# Autodesk Inventor assembly: Handle_Assembly
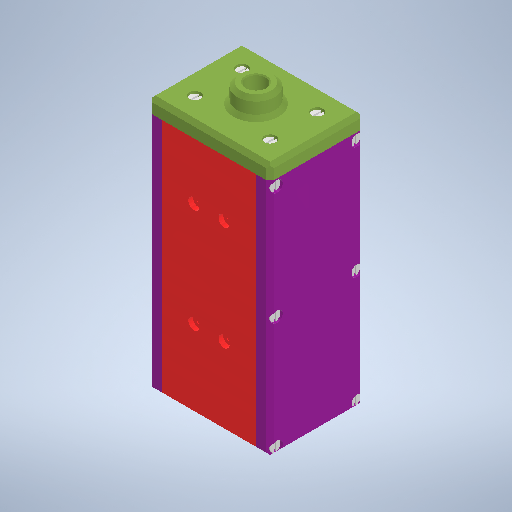
[picture p0: Inventor's stored thumbnail of the model, 512x512]
Saved by Autodesk Inventor 2026.2 (Build 302298010, 298A)
## iProperties
Created: 2026-05-07
Part Number: Handle_Assembly
Document SubType Name: Assembly
Designer: piete
Author: piete
## Documents named in this file (9)
- C:\Users\piete\Desktop\Skripsie\Documents\Detail Design\Handle Design\Handle_Assembly.iam
- C:\Users\piete\Desktop\Skripsie\Documents\Detail Design\Handle Design\Main_Cover.ipt
- C:\Users\piete\Desktop\Skripsie\Documents\Detail Design\Handle Design\Front_Cover.ipt
- C:\Users\piete\Desktop\Skripsie\Documents\Detail Design\Handle Design\Top_Covers.ipt
- C:\Users\piete\Desktop\Skripsie\Documents\Detail Design\Handle Design\Heat_Inserts.ipt
- C:\Users\piete\OneDrive\Documents\Inventor\Content Center Files\R2026\en-US\ISO 2009(2)\ISO 2009 - M3 x 20 - 17,35 - ISO.ipt
- C:\Users\piete\OneDrive\Documents\Inventor\Content Center Files\R2026\en-US\ISO 4036(2)\ISO 4036 - M3(2).ipt
- C:\Users\piete\OneDrive\Documents\Inventor\Content Center Files\R2026\en-US\ISO 2009(2)\ISO 2009 - M3 x 10 - 7,35 - ISO.ipt
- C:\Users\piete\Desktop\Skripsie\Documents\Detail Design\RS Components\186106 QS-G1_8-4-I.ipt
## Components (38 placed, 8 different names)
1. Main_Cover:1 — Mate:4, Mate:5, Mate:6, Flush:1, Mate:8, Flush:2, Mate:9, Flush:8, Mate:11, Mate:12, Mate:13, Mate:14, Mate:15, Mate:16, Flush:14, Mate:17, Mate:18, Mate:19, Mate:20, Mate:21, Mate:22, Mate:28, Mate:30, Mate:32, Mate:34, Mate:47, Mate:48, Mate:49, Mate:50
2. Front_Cover:1 — Mate:4, Mate:5, Mate:6, Mate:7, Mate:10, Mate:23, Mate:24, Mate:25, Mate:26, Flush:15, Flush:16, Flush:17, Flush:18, Angle:1, Angle:2
3. Top_Covers:1 — Flush:2, Mate:9, Mate:10, Mate:35, Mate:36, Mate:37, Mate:38, Mate:39, Mate:40, Flush:26
4. Top_Covers:2 — Flush:1, Mate:7, Mate:8, Flush:32, Mate:41, Mate:42, Mate:43, Mate:44, Mate:45, Mate:46
5. Heat_Inserts:1 — Flush:7, Flush:8, Mate:14
6. Heat_Inserts:2 — Flush:6, Flush:7, Mate:16
7. Heat_Inserts:3 — Flush:5, Flush:6, Mate:15
8. Heat_Inserts:4 — Flush:4, Flush:5, Mate:12
9. Heat_Inserts:5 — Flush:3, Mate:11
10. Heat_Inserts:6 — Flush:3, Flush:4, Mate:13
11. Heat_Inserts:7 — Flush:10, Mate:17
12. Heat_Inserts:8 — Flush:11, Mate:18
13. Heat_Inserts:9 — Flush:12, Flush:13, Mate:22
14. Heat_Inserts:10 — Flush:9, Flush:11, Flush:14, Mate:20
15. Heat_Inserts:11 — Flush:9, Flush:10, Flush:12, Mate:19
16. Heat_Inserts:12 — Flush:13, Mate:21
17. ISO 2009 M3 x 20 x 17,35:1 — Mate:25, Flush:15, Flush:20, Mate:33
18. ISO 2009 M3 x 20 x 17,35:2 — Mate:24, Flush:18, Flush:19, Angle:2, Mate:29
19. ISO 2009 M3 x 20 x 17,35:3 — Mate:26, Flush:16, Flush:20, Angle:1, Mate:31
20. ISO 2009 M3 x 20 x 17,35:4 — Mate:23, Flush:17, Flush:19, Mate:27
21. ISO 4036 M3:1 — Mate:27, Mate:28
22. ISO 4036 M3:2 — Mate:29, Mate:30
23. ISO 4036 M3:3 — Mate:31, Mate:32
24. ISO 4036 M3:4 — Mate:33, Mate:34
25. ISO 2009 M3 x 10 x 7,35:1 — Flush:25, Mate:35
26. ISO 2009 M3 x 10 x 7,35:2 — Flush:23, Mate:38
27. ISO 2009 M3 x 10 x 7,35:3 — Flush:21, Mate:39
28. ISO 2009 M3 x 10 x 7,35:4 — Flush:21, Flush:22, Mate:40, Flush:26
29. ISO 2009 M3 x 10 x 7,35:5 — Flush:22, Flush:23, Flush:24, Flush:25, Mate:37
30. ISO 2009 M3 x 10 x 7,35:6 — Flush:24, Mate:36
31. ISO 2009 M3 x 10 x 7,35:7 — Flush:31, Flush:32, Mate:42
32. ISO 2009 M3 x 10 x 7,35:8 — Flush:30, Flush:31, Mate:41
33. ISO 2009 M3 x 10 x 7,35:9 — Flush:29, Flush:30, Mate:43
34. ISO 2009 M3 x 10 x 7,35:10 — Flush:28, Flush:29, Mate:44
35. ISO 2009 M3 x 10 x 7,35:11 — Flush:27, Flush:28, Mate:46
36. ISO 2009 M3 x 10 x 7,35:12 — Flush:27, Mate:45
37. 186106 QS-G1_8-4-I:1 — Mate:48, Mate:50
38. 186106 QS-G1_8-4-I:2 — Mate:47, Mate:49
## Relationships (81: Mate 47, Flush 32, Angle 2)
- Mate:4: Main_Cover:1 ↔ Front_Cover:1
- Mate:5: Main_Cover:1 ↔ Front_Cover:1
- Mate:6: Main_Cover:1 ↔ Front_Cover:1
- Flush:1: Main_Cover:1 ↔ Top_Covers:2
- Mate:7: Front_Cover:1 ↔ Top_Covers:2
- Mate:8: Main_Cover:1 ↔ Top_Covers:2
- Flush:2: Main_Cover:1 ↔ Top_Covers:1
- Mate:9: Main_Cover:1 ↔ Top_Covers:1
- Mate:10: Front_Cover:1 ↔ Top_Covers:1
- Flush:3: Heat_Inserts:5 ↔ Heat_Inserts:6
- Flush:4: Heat_Inserts:4 ↔ Heat_Inserts:6
- Flush:5: Heat_Inserts:3 ↔ Heat_Inserts:4
- Flush:6: Heat_Inserts:2 ↔ Heat_Inserts:3
- Flush:7: Heat_Inserts:1 ↔ Heat_Inserts:2
- Flush:8: Main_Cover:1 ↔ Heat_Inserts:1
- Mate:11: Main_Cover:1 ↔ Heat_Inserts:5
- Mate:12: Main_Cover:1 ↔ Heat_Inserts:4
- Mate:13: Main_Cover:1 ↔ Heat_Inserts:6
- Mate:14: Main_Cover:1 ↔ Heat_Inserts:1
- Mate:15: Main_Cover:1 ↔ Heat_Inserts:3
- Mate:16: Main_Cover:1 ↔ Heat_Inserts:2
- Flush:9: Heat_Inserts:10 ↔ Heat_Inserts:11
- Flush:10: Heat_Inserts:7 ↔ Heat_Inserts:11
- Flush:11: Heat_Inserts:8 ↔ Heat_Inserts:10
- Flush:12: Heat_Inserts:9 ↔ Heat_Inserts:11
- Flush:13: Heat_Inserts:9 ↔ Heat_Inserts:12
- Flush:14: Main_Cover:1 ↔ Heat_Inserts:10
- Mate:17: Main_Cover:1 ↔ Heat_Inserts:7
- Mate:18: Main_Cover:1 ↔ Heat_Inserts:8
- Mate:19: Main_Cover:1 ↔ Heat_Inserts:11
- Mate:20: Main_Cover:1 ↔ Heat_Inserts:10
- Mate:21: Main_Cover:1 ↔ Heat_Inserts:12
- Mate:22: Main_Cover:1 ↔ Heat_Inserts:9
- Mate:23: Front_Cover:1 ↔ ISO 2009 M3 x 20 x 17,35:4
- Mate:24: Front_Cover:1 ↔ ISO 2009 M3 x 20 x 17,35:2
- Mate:25: Front_Cover:1 ↔ ISO 2009 M3 x 20 x 17,35:1
- Mate:26: Front_Cover:1 ↔ ISO 2009 M3 x 20 x 17,35:3
- Flush:15 (1 mm): Front_Cover:1 ↔ ISO 2009 M3 x 20 x 17,35:1
- Flush:16 (1 mm): Front_Cover:1 ↔ ISO 2009 M3 x 20 x 17,35:3
- Flush:17 (1 mm): Front_Cover:1 ↔ ISO 2009 M3 x 20 x 17,35:4
- Flush:18 (1 mm): Front_Cover:1 ↔ ISO 2009 M3 x 20 x 17,35:2
- Flush:19: ISO 2009 M3 x 20 x 17,35:2 ↔ ISO 2009 M3 x 20 x 17,35:4
- Flush:20: ISO 2009 M3 x 20 x 17,35:1 ↔ ISO 2009 M3 x 20 x 17,35:3
- Angle:1 (90 deg): Front_Cover:1 ↔ ISO 2009 M3 x 20 x 17,35:3
- Angle:2 (90 deg): Front_Cover:1 ↔ ISO 2009 M3 x 20 x 17,35:2
- Mate:27: ISO 2009 M3 x 20 x 17,35:4 ↔ ISO 4036 M3:1
- Mate:28: Main_Cover:1 ↔ ISO 4036 M3:1
- Mate:29: ISO 2009 M3 x 20 x 17,35:2 ↔ ISO 4036 M3:2
- Mate:30: Main_Cover:1 ↔ ISO 4036 M3:2
- Mate:31: ISO 2009 M3 x 20 x 17,35:3 ↔ ISO 4036 M3:3
- Mate:32: Main_Cover:1 ↔ ISO 4036 M3:3
- Mate:33: ISO 2009 M3 x 20 x 17,35:1 ↔ ISO 4036 M3:4
- Mate:34: Main_Cover:1 ↔ ISO 4036 M3:4
- Flush:21: ISO 2009 M3 x 10 x 7,35:3 ↔ ISO 2009 M3 x 10 x 7,35:4
- Flush:22: ISO 2009 M3 x 10 x 7,35:4 ↔ ISO 2009 M3 x 10 x 7,35:5
- Flush:23: ISO 2009 M3 x 10 x 7,35:2 ↔ ISO 2009 M3 x 10 x 7,35:5
- Flush:24: ISO 2009 M3 x 10 x 7,35:5 ↔ ISO 2009 M3 x 10 x 7,35:6
- Flush:25: ISO 2009 M3 x 10 x 7,35:1 ↔ ISO 2009 M3 x 10 x 7,35:5
- Mate:35: Top_Covers:1 ↔ ISO 2009 M3 x 10 x 7,35:1
- Mate:36: Top_Covers:1 ↔ ISO 2009 M3 x 10 x 7,35:6
- Mate:37: Top_Covers:1 ↔ ISO 2009 M3 x 10 x 7,35:5
- Mate:38: Top_Covers:1 ↔ ISO 2009 M3 x 10 x 7,35:2
- Mate:39: Top_Covers:1 ↔ ISO 2009 M3 x 10 x 7,35:3
- Mate:40: Top_Covers:1 ↔ ISO 2009 M3 x 10 x 7,35:4
- Flush:26 (1 mm): Top_Covers:1 ↔ ISO 2009 M3 x 10 x 7,35:4
- Flush:27: ISO 2009 M3 x 10 x 7,35:11 ↔ ISO 2009 M3 x 10 x 7,35:12
- Flush:28: ISO 2009 M3 x 10 x 7,35:10 ↔ ISO 2009 M3 x 10 x 7,35:11
- Flush:29: ISO 2009 M3 x 10 x 7,35:9 ↔ ISO 2009 M3 x 10 x 7,35:10
- Flush:30: ISO 2009 M3 x 10 x 7,35:8 ↔ ISO 2009 M3 x 10 x 7,35:9
- Flush:31: ISO 2009 M3 x 10 x 7,35:7 ↔ ISO 2009 M3 x 10 x 7,35:8
- Flush:32 (-1 mm): Top_Covers:2 ↔ ISO 2009 M3 x 10 x 7,35:7
- Mate:41: Top_Covers:2 ↔ ISO 2009 M3 x 10 x 7,35:8
- Mate:42: Top_Covers:2 ↔ ISO 2009 M3 x 10 x 7,35:7
- Mate:43: Top_Covers:2 ↔ ISO 2009 M3 x 10 x 7,35:9
- Mate:44: Top_Covers:2 ↔ ISO 2009 M3 x 10 x 7,35:10
- Mate:45: Top_Covers:2 ↔ ISO 2009 M3 x 10 x 7,35:12
- Mate:46: Top_Covers:2 ↔ ISO 2009 M3 x 10 x 7,35:11
- Mate:47: Main_Cover:1 ↔ 186106 QS-G1_8-4-I:2
- Mate:48: Main_Cover:1 ↔ 186106 QS-G1_8-4-I:1
- Mate:49: Main_Cover:1 ↔ 186106 QS-G1_8-4-I:2
- Mate:50: Main_Cover:1 ↔ 186106 QS-G1_8-4-I:1
